# Autodesk Inventor assembly: halfdrivetrain
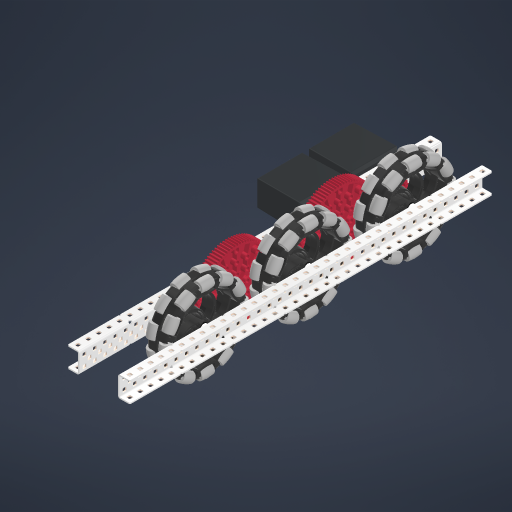
[picture p0: Inventor's stored thumbnail of the model, 512x512]
Saved by Autodesk Inventor 2023 (Build 270158000, 158)
## iProperties
Created: 2023-02-25
Part Number: halfdrivetrain
Document SubType Name: Assembly
Designer: Windows Macbook
Author: Windows Macbook
## Documents named in this file (12)
- C:\Users\Windows Macbook\Desktop\VRC-SPIN-UP\Inventor\Assembly\Pre Worlds\halfdrivetrain.iam
- C:\Users\Windows Macbook\Desktop\VRC-SPIN-UP\Inventor\Motion\Wheels\Omni Wheel\4 Omni, Square.iam
- C:\Users\Windows Macbook\Desktop\VRC-SPIN-UP\Inventor\Motion\Wheels\Omni Wheel.iam
- C:\Users\Windows Macbook\Desktop\VRC-SPIN-UP\Inventor\Motion\Gears\HS Gear\HS 84T Gear, Square.iam
- C:\Users\Windows Macbook\Desktop\VRC-SPIN-UP\Inventor\Motion\Gears\HS Gear.iam
- C:\Users\Windows Macbook\Desktop\VRC-SPIN-UP\Inventor\Motion\Gears\HS Gear\HS 36T Gear, Square.iam
- C:\Users\Windows Macbook\Desktop\VRC-SPIN-UP\Inventor\Motion\Spacers\Spacer Nylon .313 OD\NSpacer .313 OD x .125.ipt
- C:\Users\Windows Macbook\Desktop\VRC-SPIN-UP\Inventor\Motion\Spacers\Spacer Nylon .313 OD.ipt
- C:\Users\Windows Macbook\Desktop\VRC-SPIN-UP\Inventor\Motion\Spacers\Spacer Nylon .313 OD\NSpacer .313 OD x .250.ipt
- C:\Users\Windows Macbook\Desktop\VRC-SPIN-UP\Inventor\Motion\Spacers\Spacer Nylon .313 OD\NSpacer .313 OD x .375.ipt
- C:\Users\Windows Macbook\Desktop\VRC-SPIN-UP\Inventor\Electronics\V5 Simple Motor.ipt
- C:\Users\Windows Macbook\Desktop\VRC-SPIN-UP\Inventor\Structure\C Channel\Aluminum 1x2x1\Alu C 1x2x1x35.ipt
## Components (23 placed, 8 different names)
1. Alu C 1x2x1x35:1
2. Alu C 1x2x1x35:2
3. 4 Omni, Square:1 [sub-assembly] — Insert:4, Insert:7
4. HS 84T Gear, Square:3 [sub-assembly] — Insert:5
5. HS 36T Gear, Square:6 [sub-assembly] — Insert:1, Insert:3
6. NSpacer .313 OD x .125:1 — Insert:1
7. NSpacer .313 OD x .250:2 — Insert:3, Insert:4
8. NSpacer .313 OD x .125:3 — Insert:5
9. NSpacer .313 OD x .375:4 — Insert:7
10. 4 Omni, Square:2 [sub-assembly]
11. HS 36T Gear, Square:7 [sub-assembly]
12. NSpacer .313 OD x .125:5
13. NSpacer .313 OD x .250:6
14. NSpacer .313 OD x .375:7
15. 4 Omni, Square:3 [sub-assembly]
16. HS 36T Gear, Square:8 [sub-assembly]
17. NSpacer .313 OD x .125:8
18. NSpacer .313 OD x .250:9
19. NSpacer .313 OD x .375:10
20. HS 84T Gear, Square:9 [sub-assembly]
21. NSpacer .313 OD x .125:11
22. V5 Simple Motor:1
23. V5 Simple Motor:2
## Relationships (26: Insert 23, Flush 2, Mate 1)
- [Mate] (47.625 mm): Alu C 1x2x1x35:1 ↔ Alu C 1x2x1x35:2
- [Flush]: Alu C 1x2x1x35:1 ↔ Alu C 1x2x1x35:2
- [Flush]: Alu C 1x2x1x35:1 ↔ Alu C 1x2x1x35:2
- Insert:1: HS 36T Gear, Square:6 ↔ NSpacer .313 OD x .125:1
- [Insert]: Alu C 1x2x1x35:1 ↔ NSpacer .313 OD x .125:1
- Insert:3: HS 36T Gear, Square:6 ↔ NSpacer .313 OD x .250:2
- Insert:4: 4 Omni, Square:1 ↔ NSpacer .313 OD x .250:2
- Insert:5: HS 84T Gear, Square:3 ↔ NSpacer .313 OD x .125:3
- [Insert]: Alu C 1x2x1x35:1 ↔ NSpacer .313 OD x .125:3
- Insert:7: 4 Omni, Square:1 ↔ NSpacer .313 OD x .375:4
- [Insert]: HS 36T Gear, Square:7 ↔ NSpacer .313 OD x .125:5
- [Insert]: HS 36T Gear, Square:7 ↔ NSpacer .313 OD x .250:6
- [Insert]: 4 Omni, Square:2 ↔ NSpacer .313 OD x .250:6
- [Insert]: 4 Omni, Square:2 ↔ NSpacer .313 OD x .375:7
- [Insert]: HS 36T Gear, Square:8 ↔ NSpacer .313 OD x .125:8
- [Insert]: HS 36T Gear, Square:8 ↔ NSpacer .313 OD x .250:9
- [Insert]: 4 Omni, Square:3 ↔ NSpacer .313 OD x .250:9
- [Insert]: 4 Omni, Square:3 ↔ NSpacer .313 OD x .375:10
- [Insert]: Alu C 1x2x1x35:1 ↔ NSpacer .313 OD x .125:8
- [Insert]: HS 84T Gear, Square:9 ↔ NSpacer .313 OD x .125:11
- [Insert]: Alu C 1x2x1x35:1 ↔ NSpacer .313 OD x .125:11
- [Insert]: Alu C 1x2x1x35:1 ↔ NSpacer .313 OD x .125:5
- [Insert]: Alu C 1x2x1x35:1 ↔ V5 Simple Motor:1
- [Insert]: Alu C 1x2x1x35:1 ↔ V5 Simple Motor:1
- [Insert]: Alu C 1x2x1x35:1 ↔ V5 Simple Motor:2
- [Insert]: Alu C 1x2x1x35:1 ↔ V5 Simple Motor:2
## Named parameters: d13_d6 = 0 mm, d14_d8 = 0 mm, d15_d9 = 0 mm, d16_d12 = 0 mm, d17_d6 = 0 mm, d18_d8 = 0 mm, d19_d9 = 0 mm, d20_d12 = 0 mm, d22_d10 = 0 mm
